# Autodesk Inventor assembly: COMPLETE_all_parts
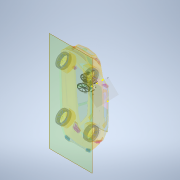
[picture p0: Inventor's stored thumbnail of the model, 180x180]
Saved by Autodesk Inventor 2021 (Build 250183000, 183)
## iProperties
Created: 2021-05-05
Part Number: COMPLETE_all_parts
Document SubType Name: Assembly
## Documents named in this file (5)
- C:\Users\ocon0143\OneDrive - Flinders\Advn Mech Design Shared\6_Development\2_Design\inventor\COMPLETE_car_Large.iam
- C:\Users\ocon0143\OneDrive - Flinders\Advn Mech Design Shared\6_Development\2_Design\inventor\vehicle_wheelchair\mb_gls\ext_GLS Assembly.iam
- C:\Users\ocon0143\OneDrive - Flinders\Advn Mech Design Shared\6_Development\2_Design\inventor\vehicle_wheelchair\wheelchair\wheelchair_box_extended.ipt
- C:\Users\ocon0143\OneDrive - Flinders\Advn Mech Design Shared\6_Development\2_Design\inventor\securing_mechanism\wheelchair_secure_devices.iam
- C:\Users\ocon0143\OneDrive - Flinders\Advn Mech Design Shared\6_Development\2_Design\inventor\securing_mechanism\secure_to_hoop_bought.ipt
## Components (4 placed, 4 different names)
1. ext_GLS Assembly:1 [sub-assembly] — Flush:1, Angle:1, Flush:2, Flush:3
2. wheelchair_box_extended:1
3. wheelchair_secure_devices:1 [sub-assembly] — Flush:7
4. secure_to_hoop_bought:1 — Flush:7
## Relationships (5: Flush 4, Angle 1)
- Flush:1: ext_GLS Assembly:1
- Angle:1 (0 deg): ext_GLS Assembly:1
- Flush:2: ext_GLS Assembly:1
- Flush:3: ext_GLS Assembly:1
- Flush:7: wheelchair_secure_devices:1 ↔ secure_to_hoop_bought:1
